# Autodesk Inventor assembly: NC1
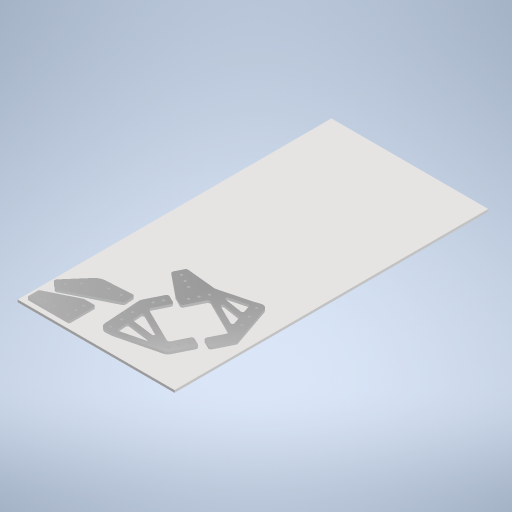
[picture p0: Inventor's stored thumbnail of the model, 512x512]
Saved by Autodesk Inventor 2023 (Build 270158000, 158)
## iProperties
Created: 2022-04-13
Part Number: NC1
Document SubType Name: Assembly
Designer: yuta
Author: yuta
## Documents named in this file (6)
- C:\Users\yuta\Desktop\R2_version1\NC1.iam
- C:\Users\yuta\Documents\NHK\NC.port.ipt
- C:\Users\yuta\Desktop\R2_version1\NC\オムニ_koteigu.ipt
- C:\Users\yuta\Desktop\R2_version1\NC\オムニ_固定具1-1.ipt
- C:\Users\yuta\Desktop\R2_version1\NC\オムニ_前1側板.ipt
- C:\Users\yuta\Desktop\R2_version1\NC\オムニ_後ろ側板.ipt
## Components (5 placed, 5 different names)
1. NC.port:1 — メイト:1, フラッシュ:1, フラッシュ:2, メイト:2, メイト:4, メイト:5, メイト:7
2. オムニ_koteigu:1 — メイト:1, フラッシュ:1, フラッシュ:2, メイト:3
3. オムニ_固定具1-1:2 — メイト:2, メイト:3, メイト:4, メイト:6
4. オムニ_前1側板:1 — メイト:5, メイト:6, メイト:8
5. オムニ_後ろ側板:2 — メイト:7, メイト:8
## Relationships (10: Mate 8, Flush 2)
- メイト:1 [Mate]: NC.port:1 ↔ オムニ_koteigu:1
- フラッシュ:1 [Flush] (6 mm): NC.port:1 ↔ オムニ_koteigu:1
- フラッシュ:2 [Flush] (6 mm): NC.port:1 ↔ オムニ_koteigu:1
- メイト:2 [Mate]: NC.port:1 ↔ オムニ_固定具1-1:2
- メイト:3 [Mate] (6 mm): オムニ_koteigu:1 ↔ オムニ_固定具1-1:2
- メイト:4 [Mate] (-8 mm): NC.port:1 ↔ オムニ_固定具1-1:2
- メイト:5 [Mate]: NC.port:1 ↔ オムニ_前1側板:1
- メイト:6 [Mate] (8 mm): オムニ_固定具1-1:2 ↔ オムニ_前1側板:1
- メイト:7 [Mate]: NC.port:1 ↔ オムニ_後ろ側板:2
- メイト:8 [Mate] (8 mm): オムニ_前1側板:1 ↔ オムニ_後ろ側板:2
